# Autodesk Inventor assembly: back_box_asembly
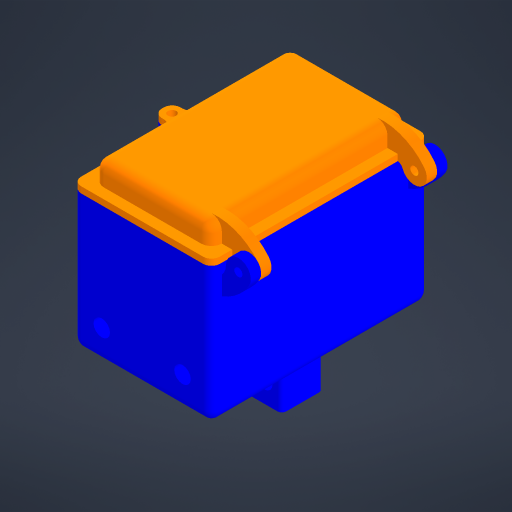
[picture p0: Inventor's stored thumbnail of the model, 512x512]
Saved by Autodesk Inventor 2024 (Build 280153000, 153)
## iProperties
Created: 2023-05-15
Part Number: back_box_asembly
Document SubType Name: Assembly
Designer: user
Author: user
## Documents named in this file (4)
- D:\Docs\Robot\3d\machine_body\back_box_asembly.iam
- D:\Docs\Robot\3d\machine_body\back_box_asembly\back_box.ipt
- D:\Docs\Robot\3d\electronics\Battery_18650_asembly.iam
- D:\Docs\Robot\3d\machine_body\back_box_asembly\back_box_cup.ipt
## Components (3 placed, 3 different names)
1. back_box:1 — Совмещение:1, Совмещение:2, Совмещение:3, Совмещение:4, Совмещение:5, Касательность:1, Касательность:2, Касательность:3, Заподлицо:1, Заподлицо:2, Заподлицо:3
2. Battery_18650_asembly:1 [sub-assembly] — Совмещение:5, Касательность:1, Касательность:2, Касательность:3
3. back_box_cup:1 — Заподлицо:1, Заподлицо:2, Заподлицо:3
## Relationships (11: Mate 5, Tangent 3, Flush 3)
- Совмещение:1 [Mate]: back_box:1
- Совмещение:2 [Mate]: back_box:1
- Совмещение:3 [Mate]: back_box:1
- Совмещение:4 [Mate]: back_box:1
- Совмещение:5 [Mate] (3 mm): back_box:1 ↔ Battery_18650_asembly:1
- Касательность:1 [Tangent]: back_box:1 ↔ Battery_18650_asembly:1
- Касательность:2 [Tangent] (1 mm): back_box:1 ↔ Battery_18650_asembly:1
- Касательность:3 [Tangent] (1 mm): back_box:1 ↔ Battery_18650_asembly:1
- Заподлицо:1 [Flush]: back_box:1 ↔ back_box_cup:1
- Заподлицо:2 [Flush]: back_box:1 ↔ back_box_cup:1
- Заподлицо:3 [Flush]: back_box:1 ↔ back_box_cup:1
